# Autodesk Inventor assembly: OCT_Probe_Asm
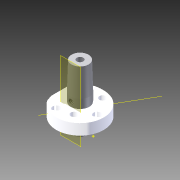
[picture p0: Inventor's stored thumbnail of the model, 180x180]
Saved by Autodesk Inventor 2011 SP2 (Build 150309200, 309)
## iProperties
Created: 2012-04-17
Part Number: OCT_Probe_Asm
Document SubType Name: Assembly
Designer: sungwook
Author: sungwook
## Documents named in this file (7)
- C:\Users\sungwook\Documents\Inventor\Micron22_top_adj_02082013\OCT Probes\OCT_Probe_Asm.iam
- C:\Users\sungwook\Documents\Inventor\Micron22_top_adj_02082013\OCT Probes\OCT_tubing_25G.ipt
- C:\Users\sungwook\Documents\Inventor\Micron22_top_adj_02082013\OCT Probes\OCT_tubing_21G.ipt
- C:\Users\sungwook\Documents\Inventor\Micron22_top_adj_02082013\OCT Probes\OCT_tubing_19G.ipt
- C:\Users\sungwook\Documents\Inventor\Micron22_top_adj_02082013\OCT Probes\OCT_tubing_17G.ipt
- C:\Users\sungwook\Documents\Inventor\Micron22_top_adj_02082013\Parts\Tool\Tool_Mount_Luer_Adapter.ipt
- C:\Users\sungwook\Documents\Inventor\Micron22_top_adj_02082013\Parts\Tool\Tool Mount_Rev.ipt
## Components (6 placed, 6 different names)
1. Tool_Mount_Luer_Adapter:1 — Mate:4, Mate:5, Mate:6, Mate:8, Mate:11, Flush:7, Mate:12, Mate:13
2. Tool Mount_Rev:1 — Mate:12, Mate:13, Angle:1
3. OCT_tubing_25G:1 — Mate:1, Mate:4, Mate:5, Mate:6, Mate:9, Mate:10
4. OCT_tubing_21G:1 — Mate:1, Mate:2, Flush:4, Mate:9, Flush:5
5. OCT_tubing_19G:1 — Mate:2, Flush:4, Flush:5, Flush:6
6. OCT_tubing_17G:1 — Mate:10, Flush:6, Mate:11, Flush:7
## Relationships (16: Mate 11, Flush 4, Angle 1)
- Mate:1: OCT_tubing_25G:1 ↔ OCT_tubing_21G:1
- Mate:2: OCT_tubing_21G:1 ↔ OCT_tubing_19G:1
- Mate:4: Tool_Mount_Luer_Adapter:1 ↔ OCT_tubing_25G:1
- Mate:5 (-50 mm): Tool_Mount_Luer_Adapter:1 ↔ OCT_tubing_25G:1
- Flush:4 (10 mm): OCT_tubing_21G:1 ↔ OCT_tubing_19G:1
- Mate:6 (-50.382 mm): Tool_Mount_Luer_Adapter:1 ↔ OCT_tubing_25G:1
- Mate:8: Tool_Mount_Luer_Adapter:1
- Mate:9: OCT_tubing_25G:1 ↔ OCT_tubing_21G:1
- Flush:5: OCT_tubing_21G:1 ↔ OCT_tubing_19G:1
- Mate:10: OCT_tubing_25G:1 ↔ OCT_tubing_17G:1
- Flush:6: OCT_tubing_19G:1 ↔ OCT_tubing_17G:1
- Mate:11: Tool_Mount_Luer_Adapter:1 ↔ OCT_tubing_17G:1
- Flush:7: Tool_Mount_Luer_Adapter:1 ↔ OCT_tubing_17G:1
- Mate:12: Tool_Mount_Luer_Adapter:1 ↔ Tool Mount_Rev:1
- Mate:13: Tool_Mount_Luer_Adapter:1 ↔ Tool Mount_Rev:1
- Angle:1 (180 deg): Tool Mount_Rev:1
